# Autodesk Inventor assembly: Assembly1
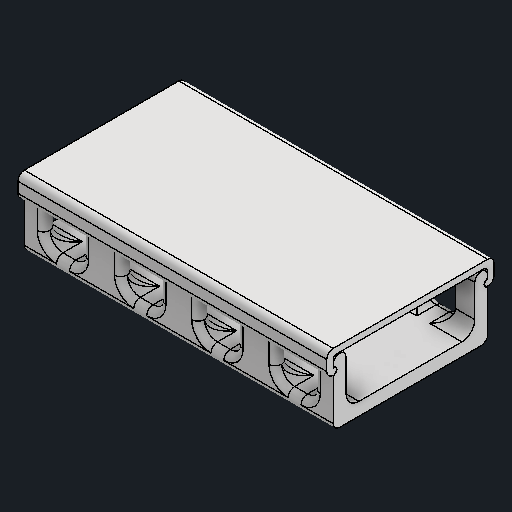
[picture p0: Inventor's stored thumbnail of the model, 512x512]
Saved by Autodesk Inventor 2026.2 (Build 302298000, 298)
## iProperties
Created: 2026-06-14
Part Number: Assembly1
Document SubType Name: Assembly
Designer: JoshuaEah
Author: JoshuaEah
## Documents named in this file (3)
- C:\Users\JoshuaEah\Documents\GitHub\Designed-Trinkets\Desktop Organization\Assembly1.iam
- C:\Users\JoshuaEah\Documents\GitHub\Designed-Trinkets\Desktop Organization\Cable Duct.ipt
- C:\Users\JoshuaEah\Documents\GitHub\Designed-Trinkets\Desktop Organization\Duct Cover.ipt
## Components (2 placed, 2 different names)
1. Cable Duct:1 — Mate:1, Mate:2, Flush:1
2. Duct Cover:1 — Mate:1, Mate:2, Flush:1
## Relationships (3: Mate 2, Flush 1)
- Mate:1: Cable Duct:1 ↔ Duct Cover:1
- Mate:2: Cable Duct:1 ↔ Duct Cover:1
- Flush:1: Cable Duct:1 ↔ Duct Cover:1
